# Autodesk Inventor assembly: E006-Carter
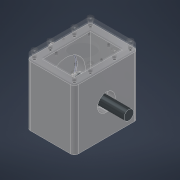
[picture p0: Inventor's stored thumbnail of the model, 180x180]
Saved by Autodesk Inventor 2021.3 (Build 253353000, 353)
## iProperties
Created: 2022-04-01
Part Number: E006-Carter
Document SubType Name: Assembly
Designer: remi
Author: remi
## Documents named in this file (10)
- C:\Users\remi\OneDrive\Documents\Cours\05-HEVS\S2fb\mechanic\CCo\project\Compressor\E006-Carter.iam
- C:\Users\remi\OneDrive\Documents\Cours\05-HEVS\S2fb\mechanic\CCo\project\Compressor\P016-Carter_corps.ipt
- C:\Users\remi\OneDrive\Documents\Cours\05-HEVS\S2fb\mechanic\CCo\project\Compressor\P015-Vilbrequin.ipt
- C:\Users\remi\OneDrive\Documents\Cours\05-HEVS\S2fb\mechanic\CCo\project\Compressor\P017-Carter_chapeau.ipt
- C:\Users\remi\OneDrive\Documents\Cours\05-HEVS\S2fb\mechanic\CCo\project\Compressor\P018-Joint_carter_chapeau.ipt
- C:\Users\remi\OneDrive\Documents\Cours\05-HEVS\S2fb\mechanic\CCo\project\Compressor\P020-Fixation_roulement_vilebrequin.ipt
- C:\Users\remi\OneDrive\Documents\Cours\05-HEVS\S2fb\mechanic\CCo\project\Compressor\R2021\en-US\AS 1420\AS 1420 - 1973 - M4 x 14.ipt
- C:\Users\remi\OneDrive\Documents\Cours\05-HEVS\S2fb\mechanic\CCo\project\Compressor\R2021\en-US\AS 1420\AS 1420 - 1973 - M4 x 8.ipt
- C:\Users\remi\OneDrive\Documents\Cours\05-HEVS\S2fb\mechanic\CCo\project\Compressor\P021-Bouchon_carter_vilbrequin.ipt
- C:\Users\remi\OneDrive\Documents\Cours\05-HEVS\S2fb\mechanic\CCo\project\Compressor\P022-Joint_carter_bouchon_vilbrequin.ipt
## Components (22 placed, 9 different names)
1. P016-Carter_corps:1 — Mate:3, Mate:6, Flush:1, Flush:2, Mate:9, Mate:10, Mate:11
2. P015-Vilbrequin:1 — Mate:3, Mate:7, Mate:8
3. P017-Carter_chapeau:1 — Mate:4, Mate:5, Flush:1, Flush:2, Insert:1, Insert:2, Insert:3, Insert:4, Insert:5, Insert:6, Insert:7, Insert:8
4. P018-Joint_carter_chapeau:1 — Mate:4, Mate:5, Mate:6
5. P020-Fixation_roulement_vilebrequin:1 — Mate:7, Mate:8, Insert:9
6. P021-Bouchon_carter_vilbrequin:1 — Mate:9, Insert:10, Insert:11, Insert:12, Insert:13, Insert:14, Insert:15
7. P022-Joint_carter_bouchon_vilbrequin:1 — Mate:10, Mate:11
8. AS 1420 - Metric M4 x 8:2 — Insert:10
9. AS 1420 - Metric M4 x 8:3 — Insert:11
10. AS 1420 - Metric M4 x 8:4 — Insert:12
11. AS 1420 - Metric M4 x 8:5 — Insert:13
12. AS 1420 - Metric M4 x 8:6 — Insert:14
13. AS 1420 - Metric M4 x 8:7 — Insert:15
14. AS 1420 - Metric M4 x 14:1 — Insert:1
15. AS 1420 - Metric M4 x 14:2 — Insert:2
16. AS 1420 - Metric M4 x 14:3 — Insert:3
17. AS 1420 - Metric M4 x 14:4 — Insert:4
18. AS 1420 - Metric M4 x 14:5 — Insert:5
19. AS 1420 - Metric M4 x 14:6 — Insert:6
20. AS 1420 - Metric M4 x 14:7 — Insert:7
21. AS 1420 - Metric M4 x 14:8 — Insert:8
22. AS 1420 - Metric M4 x 8:1 — Insert:9
## Relationships (26: Insert 15, Mate 9, Flush 2)
- Mate:3: P016-Carter_corps:1 ↔ P015-Vilbrequin:1
- Mate:4: P017-Carter_chapeau:1 ↔ P018-Joint_carter_chapeau:1
- Mate:5: P017-Carter_chapeau:1 ↔ P018-Joint_carter_chapeau:1
- Mate:6: P016-Carter_corps:1 ↔ P018-Joint_carter_chapeau:1
- Flush:1: P016-Carter_corps:1 ↔ P017-Carter_chapeau:1
- Flush:2: P016-Carter_corps:1 ↔ P017-Carter_chapeau:1
- Mate:7: P015-Vilbrequin:1 ↔ P020-Fixation_roulement_vilebrequin:1
- Mate:8: P015-Vilbrequin:1 ↔ P020-Fixation_roulement_vilebrequin:1
- Insert:1: P017-Carter_chapeau:1 ↔ AS 1420 - Metric M4 x 14:1
- Insert:2: P017-Carter_chapeau:1 ↔ AS 1420 - Metric M4 x 14:2
- Insert:3: P017-Carter_chapeau:1 ↔ AS 1420 - Metric M4 x 14:3
- Insert:4: P017-Carter_chapeau:1 ↔ AS 1420 - Metric M4 x 14:4
- Insert:5: P017-Carter_chapeau:1 ↔ AS 1420 - Metric M4 x 14:5
- Insert:6: P017-Carter_chapeau:1 ↔ AS 1420 - Metric M4 x 14:6
- Insert:7: P017-Carter_chapeau:1 ↔ AS 1420 - Metric M4 x 14:7
- Insert:8: P017-Carter_chapeau:1 ↔ AS 1420 - Metric M4 x 14:8
- Insert:9: P020-Fixation_roulement_vilebrequin:1 ↔ AS 1420 - Metric M4 x 8:1
- Mate:9 (2 mm): P016-Carter_corps:1 ↔ P021-Bouchon_carter_vilbrequin:1
- Mate:10: P016-Carter_corps:1 ↔ P022-Joint_carter_bouchon_vilbrequin:1
- Mate:11: P016-Carter_corps:1 ↔ P022-Joint_carter_bouchon_vilbrequin:1
- Insert:10: P021-Bouchon_carter_vilbrequin:1 ↔ AS 1420 - Metric M4 x 8:2
- Insert:11: P021-Bouchon_carter_vilbrequin:1 ↔ AS 1420 - Metric M4 x 8:3
- Insert:12: P021-Bouchon_carter_vilbrequin:1 ↔ AS 1420 - Metric M4 x 8:4
- Insert:13: P021-Bouchon_carter_vilbrequin:1 ↔ AS 1420 - Metric M4 x 8:5
- Insert:14: P021-Bouchon_carter_vilbrequin:1 ↔ AS 1420 - Metric M4 x 8:6
- Insert:15: P021-Bouchon_carter_vilbrequin:1 ↔ AS 1420 - Metric M4 x 8:7
